# Autodesk Inventor assembly: Bumper Attachment Assembly
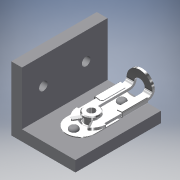
[picture p0: Inventor's stored thumbnail of the model, 180x180]
Saved by Autodesk Inventor 2019 (Build 230136000, 136)
## iProperties
Created: 2018-11-17
Part Number: Bumper Attachment Assembly
Document SubType Name: Assembly
Designer: maste
Author: maste
## Documents named in this file (5)
- D:\Summer Drive Base V1\Summer Drivebase\Bumper Attachment Assembly.iam
- D:\Summer Drive Base V1\Summer Drivebase\Bumper L-Bracket.ipt
- D:\Summer Drive Base V1\Summer Drivebase\1872A720_SLIDE-SNAP DRAW LATCH.ipt
- D:\Summer Drive Base V1\Summer Drivebase\0.125in Rivet.ipt
- D:\Summer Drive Base V1\Summer Drivebase\Bumper Attachment Spacer.ipt
## Components (5 placed, 4 different names)
1. Bumper L-Bracket:1 — Mate:1, Mate:2, Mate:3
2. 1872A720_SLIDE-SNAP DRAW LATCH:1 — Mate:1, Mate:2, Mate:3, Mate:4, Mate:5, Mate:6, Mate:7, Rotation:1, Rotation:2, Mate:8, Mate:9, Rotation:3
3. 0.125in Rivet:1 — Mate:5, Mate:7, Rotation:1
4. 0.125in Rivet:2 — Mate:4, Mate:6, Rotation:2
5. Bumper Attachment Spacer:1 — Mate:8, Mate:9, Rotation:3
## Relationships (12: Mate 9, RelateRotation 3)
- Mate:1: Bumper L-Bracket:1 ↔ 1872A720_SLIDE-SNAP DRAW LATCH:1
- Mate:2: Bumper L-Bracket:1 ↔ 1872A720_SLIDE-SNAP DRAW LATCH:1
- Mate:3: Bumper L-Bracket:1 ↔ 1872A720_SLIDE-SNAP DRAW LATCH:1
- Mate:4: 1872A720_SLIDE-SNAP DRAW LATCH:1 ↔ 0.125in Rivet:2
- Mate:5: 1872A720_SLIDE-SNAP DRAW LATCH:1 ↔ 0.125in Rivet:1
- Mate:6: 1872A720_SLIDE-SNAP DRAW LATCH:1 ↔ 0.125in Rivet:2
- Mate:7: 1872A720_SLIDE-SNAP DRAW LATCH:1 ↔ 0.125in Rivet:1
- Rotation:1 [RelateRotation] (1 ul): 1872A720_SLIDE-SNAP DRAW LATCH:1 ↔ 0.125in Rivet:1
- Rotation:2 [RelateRotation] (1 ul): 1872A720_SLIDE-SNAP DRAW LATCH:1 ↔ 0.125in Rivet:2
- Mate:8: 1872A720_SLIDE-SNAP DRAW LATCH:1 ↔ Bumper Attachment Spacer:1
- Mate:9: 1872A720_SLIDE-SNAP DRAW LATCH:1 ↔ Bumper Attachment Spacer:1
- Rotation:3 [RelateRotation] (1 ul): 1872A720_SLIDE-SNAP DRAW LATCH:1 ↔ Bumper Attachment Spacer:1
